# Autodesk Inventor assembly: GEABA1.0-80-10-B-12
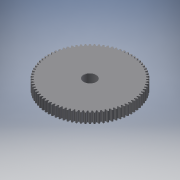
[picture p0: Inventor's stored thumbnail of the model, 180x180]
Saved by Autodesk Inventor 2019 (Build 230136000, 136)
## iProperties
Category: PARTsolutions
Company: MISUMI
Created: 2022-11-02
Part Number: GEABA1.0-80-10-B-12
Catalog Web Link: www.cadenas.de
Description: GEABM, GEABMS, GEABMT, GEABP, GEABPS, GEABPT, GEABA, GEABAS, GEABAT-Plastic Spur Gears - Pressure Angle 20 Degrees, Module 0.5/0.8/1.0/1.5/2.0/2.5/3.0
Vendor: MISUMI
Document SubType Name: Assembly
Designer: psAdmin
Manufacturer: MISUMI
Mass: 60.2372 g
Surface Area: 168.492 cm^2
Volume: 60.2372 cm^3
Density: 1 g/cm^3
Title: GEABA1.0-80-10-B-12
Author: Cadenas PARTsolutions
Comments: Plastic Spur Gears - Pressure Angle 20 Degrees, Module 0.5/0.8/1.0/1.5/2.0/2.5/3.0
PSOL_IDENT_0: {$CADENAS_DATA/23d-libs/misumi/metric/54_spur_gears/geabms20_asmtab.prj},397 {VTYP=3D},{STYP=ASSTAB}
PSOL_IDENT_1: ,{NB=GEABA1.0-80-10-B-12},{LINA=GEABA1.0-80-10-B-12},{NN=GEABM, GEABMS, GEABMT, GEABP, GEABPS, GEABP
PSOL_IDENT_2: T, GEABA, GEABAS, GEABAT},{DATE=16.08.2021 10:08:31},{GEOMDATE=16.08.2021 10:08:28},{VERSION=},{LINE
PSOL_IDENT_3: ID=30},{WBVAR=MATSG,MATCR,NT,B,TS,PS,ALT1,ALT2,TPC,ALT11,ALT10,BS,ALT3,Z,J,ALT4,Q,R,S,T,ALT5,LFC,LTC
PSOL_IDENT_4: ,MALT5,ALT6,KFC,KTC,K},{WBNUMERIC=NT,B,BS,Z,J,Q,R,S,T,LFC,LTC,KFC,KTC,K}  {NB=GEABA1.0-80-10-B-12},{
PSOL_IDENT_5: LINA=GEABA1.0-80-10-B-12},{KT=DUMMY},{PN=GEABA1.0-80-10-B-12},{TYPE=GEABA},{MATSG=PB},{MATSGALG='MCN'
PSOL_IDENT_6: ,'MC Nylon','PW','Polyacetal White','PB','Polyacetal Blue'},{MATCR=},{MATCRALG='','-','S45C','1045 C
PSOL_IDENT_7: arbon Steel','SUS304','304 Stainless Steel'},{MOD=1.0},{MOD1=1.0},{NT=80},{NTALG=15,16,18,20,22,24,2
PSOL_IDENT_8: 5,26,28,30,32,35,36,40,45,48,50,55,60,70,75,80,90,100,120},{B=10},{BALG=10,15},{TS=B},{TSALG='A','A'
PSOL_IDENT_9: ,'B','B'},{TSPN=-B},{PS=12},{PSALG='10','10','11','11','12','12','13','13','14','14','15','15','16','
PSOL_IDENT_10: 16','17','17','18','18','19','19','20','20','21','21','22','22','23','23','24','24','25','25','26','
PSOL_IDENT_11: 26','27','27','28','28'},{PSCRL='10','10','11','11','12','12','13','13','14','14','15','15','16','16'
PSOL_IDENT_12: ,'17','17','18','18','19','19','20','20','21','21','22','22','23','23','24','24','25','25','26','26'
PSOL_IDENT_13: ,'27','27','28','28'},{PSCRW='10','10','12','12','15','15','20','20'},{DD=80.0},{DD05=40},{DD08=64},
PSOL_IDENT_14: {DD10=80},{DD15=120},{DD20=0},{DD25=0},{DD30=0},{D=82.0},{D05=41},{D08=65.6},{D10=82},{D15=123},{D20=
PSOL_IDENT_15: 0},{D25=0},{D30=0},{G=77.50},{G05=38.75},{G08=62},{G10=77.5},{G15=116.25},{G20=0},{G25=0},{G30=0},{H=
PSOL_IDENT_16: 40.0},{L=20},{LL1=10},{LL2=4.0},{M=M4},{M3D=4},{P=12.00},{DD1=0},{CIFR=15},{CIFM=4},{CIFK=0},{CIFTAP=
PSOL_IDENT_17: 1},{SCREW=4.000},{SCREWL=3.000},{ALT1=},{ALT1ALG='','w/o Set Screw','KC90','with KC90 (Set Screw)','
PSOL_IDENT_18: KC120','with KC120 (Set Screw)'},{ALT1PN=},{ALT2=},{ALT2ALG='','w/o TPC (Tapped Hole Dimension)','TP
PSOL_IDENT_19: C','with TPC (Tapped Hole Dimension)'},{TPC=N/A},{TPCALG='N/A'},{ALT2PN=},{KC=0},{ALT11=},{ALT11ALG=''
PSOL_IDENT_20: , 'w/o GBA (Gear bottom adjustment of phase focus)', 'GBA', 'with GBA (Gear bottom adjustment of pha
PSOL_IDENT_21: se focus)' },{ALT11PN=},{DEG=0},{ALT10=},{ALT10ALG= '','w/o BS (Boss Cut)','BS','with BS (Boss Cut)'
PSOL_IDENT_22: },{ALT10PN=},{BS=0.0},{BSALG=0},{BSMIN=7.000},{BSMINALG=7},{BSMAX=10},{LL13D=10},{LL23D=16},{ALT3=}
PSOL_IDENT_23: ,{ALT3ALG= '','w/o Stepped Hole','DHL','with DHL (Stepped Hole)','DHR','with DHR (Stepped Hole)' },{
PSOL_IDENT_24: ALT3PN=},{ZJPN=},{ALT31=1},{ALT32=1},{Z=0},{ZALG=0},{ZMINL=14},{ZMAXL=73},{ZMINR=14},{ZMAXR=36},{ZPN=
PSOL_IDENT_25: },{J=0.0},{JALG=0},{JMIN=2},{JMAX=0},{JPN=},{ALT4=},{ALT4ALG= '','w/o WDH (Both Ends Stepped Hole)','
PSOL_IDENT_26: WDH','with WDH (Both Ends Stepped Hole)' },{ALT4PN=},{QRSTPN=},{LB=20.000},{Q=0},{QALG=0},{QMIN=14},
PSOL_IDENT_27: {QMAX=36},{QPN=},{R=0},{RALG=0},{RMIN=14},{RMAX=36},{RPN=},{S=0},{SALG=0},{SMIN=3},{SMAX=14},{SPN=},
PSOL_IDENT_28: {T=0},{TALG=0},{TMIN=3},{TMAX=0},{TPN=},{ALT5=},{ALT5ALG= '','Not applicable' },{LFC=0},{LFCALG=0},{
PSOL_IDENT_29: LTC=0},{LTCALG=0},{LPCDMIN=20},{LPCDMAX=70},{LCMAX=73},{MALT5=N/A},{MALT5ALG= 'N/A' },{LCMAX2=70},{C=
PSOL_IDENT_30: 0.0},{ALT5PN=},{ALT6=},{ALT6ALG= '','w/o Side Through Hole','KFC','with KFC (Side Through Hole)','KT
PSOL_IDENT_31: C','with KTC (Side Through Hole)' },{ALT6PN=},{KFTCPN=},{KFC=0},{KFCALG=[0]},{KFCPN=},{KTC=0},{KTCAL
PSOL_IDENT_32: G=[0]},{KTCPN=},{KPCDMIN1=19},{KPCDMAX1=33},{KPCDMIN2=47},{KPCDMAX2=70},{K=0.0},{KALG=[0]},{KPCD=0},
PSOL_IDENT_33: {KPN=},{AG=0},{LBS=20},{PCD=0},{SHN=0},{SHDEG1=0},{SHDEG2=0},{PZQRDD2=12},{PPATH=geabms20/geabms20_a
PSOL_IDENT_34: smtpl.prj}
NB: GEABA1.0-80-10-B-12
NN: GEABM, GEABMS, GEABMT, GEABP, GEABPS, GEABPT, GEABA, GEABAS, GEABAT
NT: 80
NBSYN: $PN.
LINA: GEABA1.0-80-10-B-12
CATALOG: Misumi
PN: GEABA1.0-80-10-B-12
MATSG: Polyacetal Blue
MATCR: -
MOD: 1.0
B: 10
TS: B
PS: 12
DD: 80
D: 82
G: 77.5
H: 40
L: 20
LL1: 10
LL2: 4
M: M4
DD1: 0
ALT1: w/o Set Screw
ALT2: w/o TPC (Tapped Hole Dimension)
TPC: N/A
ALT11: w/o GBA (Gear bottom adjustment of phase focus)
ALT10: w/o BS (Boss Cut)
BS: 0
ALT3: w/o Stepped Hole
Z: 0
J: 0
ALT4: w/o WDH (Both Ends Stepped Hole)
Q: 0
R: 0
S: 0
T: 0
ALT5: Not applicable
LFC: 0
LTC: 0
MALT5: N/A
C: 0
ALT6: w/o Side Through Hole
KFC: 0
KTC: 0
K: 0
SUPPLIER: MISUMI
ARTICLENO: GEABA1.0-80-10-B-12
BOMINFO: GEABA1.0-80-10-B-12
CREATOR: CADENAS GmbH
## Documents named in this file (3)
- e:\temp\worker_COMMON_3\temp\tmp_2284_54_DDGAl\format_0\GEABA1_0-80-10-B-12.iam
- e:\temp\worker_COMMON_3\temp\tmp_2284_54_DDGAl\format_0\GEABA1_0-80-10-B-12_b.ipt
- e:\temp\worker_COMMON_3\temp\tmp_2284_54_DDGAl\format_0\SET-SCREW4-3.ipt
## Components (2 placed, 2 different names)
1. GEABA1_0-80-10-B-12_b:1 — gear_to_screw_XY@1 <-> CP_XY@2, gear_to_screw_Z@1 <-> CP_Z@2, gear_to_screw_YZ@1 <-> CP_YZ@2
2. SET-SCREW4-3:1 — gear_to_screw_XY@1 <-> CP_XY@2, gear_to_screw_Z@1 <-> CP_Z@2, gear_to_screw_YZ@1 <-> CP_YZ@2
## Relationships (3: Mate 2, Angle 1)
- gear_to_screw_XY@1 <-> CP_XY@2 [Mate]: GEABA1_0-80-10-B-12_b:1 ↔ SET-SCREW4-3:1
- gear_to_screw_Z@1 <-> CP_Z@2 [Mate]: GEABA1_0-80-10-B-12_b:1 ↔ SET-SCREW4-3:1
- gear_to_screw_YZ@1 <-> CP_YZ@2 [Angle] (0 deg): GEABA1_0-80-10-B-12_b:1 ↔ SET-SCREW4-3:1
